# Autodesk Inventor assembly: WheelAssembly3.0
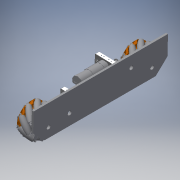
[picture p0: Inventor's stored thumbnail of the model, 180x180]
Saved by Autodesk Inventor 2017 (Build 210142000, 142)
## iProperties
Created: 2017-07-22
Part Number: WheelAssembly3.0
Document SubType Name: Assembly
Designer: User
Author: User
## Documents named in this file (6)
- C:\Robotics\CAD\WheelAssembly3.0.iam
- C:\Robotics\CAD\2016-17_CAD\DriveTrain3.0.ipt
- C:\Robotics\CAD\COTSParts\Wheels\AndyMark Mecanum Wheels\100mm Aluminum Mecanum wheels.ipt
- C:\Robotics\CAD\COTSParts\Motors\Andymark 2964  NeveRest 40 Motor.ipt
- C:\Robotics\CAD\COTSParts\Tetrix\tetrix-motor-mounts-1.snapshot.1\Tetrex 2pc motor mount.ipt
- C:\Robotics\CAD\COTSParts\Actobotics\615 parts\615398.ipt
## Components (11 placed, 5 different names)
1. DriveTrain3.0:1 — Insert:1, Insert:2, Flush:3, Flush:4, Mate:2, Flush:5, Mate:3, Flush:6, Angle:1, Insert:7, Insert:8, Angle:2
2. 100mm Aluminum Mecanum wheels:1 — Insert:2
3. 100mm Aluminum Mecanum wheels:2 — Insert:1
4. Andymark 2964  NeveRest 40 Motor:1 — Insert:3, Insert:6, Angle:2
5. Andymark 2964  NeveRest 40 Motor:2 — Insert:4, Insert:5, Angle:1
6. Tetrex 2pc motor mount:1 — Insert:3, Flush:3, Mate:3, Flush:6
7. Tetrex 2pc motor mount:2 — Insert:4, Flush:4, Mate:2, Flush:5
8. 615398:1 — Insert:5
9. 615398:2 — Insert:6
10. 615398:3 — Insert:7
11. 615398:4 — Insert:8
## Relationships (16: Insert 8, Flush 4, Mate 2, Angle 2)
- Insert:1 (8.3312 mm): DriveTrain3.0:1 ↔ 100mm Aluminum Mecanum wheels:2
- Insert:2 (8.3312 mm): DriveTrain3.0:1 ↔ 100mm Aluminum Mecanum wheels:1
- Insert:3: Andymark 2964  NeveRest 40 Motor:1 ↔ Tetrex 2pc motor mount:1
- Insert:4: Andymark 2964  NeveRest 40 Motor:2 ↔ Tetrex 2pc motor mount:2
- Flush:3 (159.5374 mm): DriveTrain3.0:1 ↔ Tetrex 2pc motor mount:1
- Flush:4 (159.5374 mm): DriveTrain3.0:1 ↔ Tetrex 2pc motor mount:2
- Insert:5: Andymark 2964  NeveRest 40 Motor:2 ↔ 615398:1
- Mate:2: DriveTrain3.0:1 ↔ Tetrex 2pc motor mount:2
- Flush:5 (7.3152 mm): DriveTrain3.0:1 ↔ Tetrex 2pc motor mount:2
- Mate:3: DriveTrain3.0:1 ↔ Tetrex 2pc motor mount:1
- Flush:6 (-20.3454 mm): DriveTrain3.0:1 ↔ Tetrex 2pc motor mount:1
- Angle:1 (0 deg): DriveTrain3.0:1 ↔ Andymark 2964  NeveRest 40 Motor:2
- Insert:6: Andymark 2964  NeveRest 40 Motor:1 ↔ 615398:2
- Insert:7 (25.4508 mm): DriveTrain3.0:1 ↔ 615398:3
- Insert:8 (25.4508 mm): DriveTrain3.0:1 ↔ 615398:4
- Angle:2 (180 deg): DriveTrain3.0:1 ↔ Andymark 2964  NeveRest 40 Motor:1
